# Autodesk Inventor assembly: E006_Boitier_v4
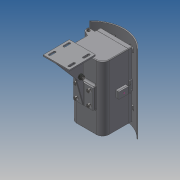
[picture p0: Inventor's stored thumbnail of the model, 180x180]
Saved by Autodesk Inventor 2021.3 (Build 253353000, 353)
## iProperties
Created: 2021-12-10
Part Number: E006_Boitier_v4
Document SubType Name: Assembly
Designer: gabri
Author: gabri
## Documents named in this file (21)
- D:\PGA\E006_Boitier_v4.iam
- D:\PGA\P037_BoitierCouvercleV4_fond.ipt
- D:\PGA\P038_BoitierCouvercleV4_couvercle.ipt
- D:\PGA\P039_BoitierCouvercleV4_capot.ipt
- D:\PGA\E003_BoitierEcran.iam
- C:\Users\gabri\Documents\Inventor\Content Center Files\R2021\en-US\AS 1474(2)\AS 1474 - M6(2).ipt
- D:\PGA\P044_SupportCaméra.ipt
- D:\PGA\P045_SupportUniversel.ipt
- C:\Users\gabri\Documents\Inventor\Content Center Files\R2021\en-US\ISO 4017(1)\ISO 4017 - M8 x 20 - ISO.ipt
- C:\Users\gabri\Documents\Inventor\Content Center Files\R2021\en-US\ISO 7040\DIEN EN ISO 7040 - M8.ipt
- D:\PGA\P046_AxeCouvercleFretté.ipt
- C:\Users\gabri\Documents\Inventor\Content Center Files\R2021\en-US\BS EN ISO 4762\BS EN ISO 4762 - M4 x 8(1).ipt
- C:\Users\gabri\Documents\Inventor\Content Center Files\R2021\en-US\DIN 6796\DIN 6796 - 4.ipt
- C:\Users\gabri\Documents\Inventor\Content Center Files\R2021\en-US\BS EN ISO 4762\BS EN ISO 4762 - M6 x 10(1).ipt
- C:\Users\gabri\Documents\Inventor\Content Center Files\R2021\en-US\BS EN ISO 4762\BS EN ISO 4762 - M5 x 16(1).ipt
- D:\PGA\P048_BoitierCouvercleV4_joint.ipt
- D:\PGA\P049_SupportTube.ipt
- D:\PGA\P050_SupportTube2.ipt
- D:\PGA\E007_Boitier_v4_moduleElectronique.iam
- D:\PGA\P051_HautGrenouillere.ipt
- D:\PGA\P052_BasGrenouillere.ipt
## Components (31 placed, 20 different names)
1. P037_BoitierCouvercleV4_fond:1 — Mate:1, Mate:2, Mate:3, Mate:5, Flush:2, Flush:3, Mate:10, Mate:11, Mate:32, Mate:33, Mate:34, Mate:35, Mate:36, Mate:37, Mate:38, Mate:39, Mate:40, Flush:4, Mate:44, Mate:58, Flush:5, Mate:59, Mate:61, Mate:64, Mate:65, Mate:69, Mate:70, Mate:71, Mate:75, Flush:7, Flush:8
2. P038_BoitierCouvercleV4_couvercle:1 — Mate:7, Mate:30, Mate:31, Insert:7, Insert:8, Insert:9, Insert:10
3. P039_BoitierCouvercleV4_capot:1 — Mate:5, Flush:2, Mate:7, Mate:30, Mate:31, Mate:72, Mate:73, Mate:74
4. E003_BoitierEcran:1 [sub-assembly] — Flush:3, Mate:10, Mate:11
5. AS 1474 (Square Nut) - Metric M6:1 — Mate:34, Mate:35
6. AS 1474 (Square Nut) - Metric M6:2 — Mate:32, Mate:33
7. AS 1474 (Square Nut) - Metric M6:3 — Mate:36, Mate:37
8. AS 1474 (Square Nut) - Metric M6:4 — Mate:38, Mate:39, Mate:41, Mate:44
9. P044_SupportCaméra:1 — Mate:40, Flush:4, Mate:41, Mate:42, Mate:43, Mate:45, Mate:46, Insert:3, Insert:4, Insert:5, Insert:6, Mate:68
10. P045_SupportUniversel:1 — Mate:42, Mate:43, Mate:48
11. ISO 4017 M8 x 20:1 — Mate:45, Mate:46, Mate:47, Mate:67
12. DIN EN ISO 7040 M8:1 — Mate:47, Mate:48
13. P046_AxeCouvercleFretté:1 — Mate:58, Flush:5, Mate:60, Mate:62
14. BS EN ISO 4762 - Metric M4 x 8:1 — Insert:2
15. BS EN ISO 4762 - Metric M4 x 8:2 — Insert:1
16. DIN 6796 4:1 — Mate:61, Mate:62, Insert:1
17. DIN 6796 4:2 — Mate:59, Mate:60, Insert:2
18. BS EN ISO 4762 - Metric M6 x 10:1 — Insert:3
19. BS EN ISO 4762 - Metric M6 x 10:2 — Insert:4
20. BS EN ISO 4762 - Metric M6 x 10:3 — Insert:5
21. BS EN ISO 4762 - Metric M6 x 10:4 — Insert:6
22. BS EN ISO 4762 - Metric M5 x 16:1 — Insert:8
23. BS EN ISO 4762 - Metric M5 x 16:2 — Insert:10
24. BS EN ISO 4762 - Metric M5 x 16:3 — Insert:9
25. BS EN ISO 4762 - Metric M5 x 16:4 — Insert:7
26. P048_BoitierCouvercleV4_joint:1 — Mate:64, Mate:65
27. P049_SupportTube:1 — Mate:66, Flush:6, Mate:67, Mate:68
28. P050_SupportTube2:1 — Mate:66, Flush:6
29. E007_Boitier_v4_moduleElectronique:1 [sub-assembly] — Mate:69, Mate:70, Mate:71
30. P051_HautGrenouillere:1 — Mate:72, Mate:73, Mate:74
31. P052_BasGrenouillere:1 — Mate:75, Flush:7, Flush:8
## Relationships (60: Mate 43, Insert 10, Flush 7)
- Mate:1: P037_BoitierCouvercleV4_fond:1
- Mate:2: P037_BoitierCouvercleV4_fond:1
- Mate:3: P037_BoitierCouvercleV4_fond:1
- Mate:5: P037_BoitierCouvercleV4_fond:1 ↔ P039_BoitierCouvercleV4_capot:1
- Flush:2: P037_BoitierCouvercleV4_fond:1 ↔ P039_BoitierCouvercleV4_capot:1
- Mate:7: P038_BoitierCouvercleV4_couvercle:1 ↔ P039_BoitierCouvercleV4_capot:1
- Flush:3: P037_BoitierCouvercleV4_fond:1 ↔ E003_BoitierEcran:1
- Mate:10: P037_BoitierCouvercleV4_fond:1 ↔ E003_BoitierEcran:1
- Mate:11: P037_BoitierCouvercleV4_fond:1 ↔ E003_BoitierEcran:1
- Mate:30: P038_BoitierCouvercleV4_couvercle:1 ↔ P039_BoitierCouvercleV4_capot:1
- Mate:31: P038_BoitierCouvercleV4_couvercle:1 ↔ P039_BoitierCouvercleV4_capot:1
- Mate:32: P037_BoitierCouvercleV4_fond:1 ↔ AS 1474 (Square Nut) - Metric M6:2
- Mate:33: P037_BoitierCouvercleV4_fond:1 ↔ AS 1474 (Square Nut) - Metric M6:2
- Mate:34: P037_BoitierCouvercleV4_fond:1 ↔ AS 1474 (Square Nut) - Metric M6:1
- Mate:35: P037_BoitierCouvercleV4_fond:1 ↔ AS 1474 (Square Nut) - Metric M6:1
- Mate:36: P037_BoitierCouvercleV4_fond:1 ↔ AS 1474 (Square Nut) - Metric M6:3
- Mate:37: P037_BoitierCouvercleV4_fond:1 ↔ AS 1474 (Square Nut) - Metric M6:3
- Mate:38: P037_BoitierCouvercleV4_fond:1 ↔ AS 1474 (Square Nut) - Metric M6:4
- Mate:39: P037_BoitierCouvercleV4_fond:1 ↔ AS 1474 (Square Nut) - Metric M6:4
- Mate:40: P037_BoitierCouvercleV4_fond:1 ↔ P044_SupportCaméra:1
- Flush:4: P037_BoitierCouvercleV4_fond:1 ↔ P044_SupportCaméra:1
- Mate:41: AS 1474 (Square Nut) - Metric M6:4 ↔ P044_SupportCaméra:1
- Mate:42: P044_SupportCaméra:1 ↔ P045_SupportUniversel:1
- Mate:43: P044_SupportCaméra:1 ↔ P045_SupportUniversel:1
- Mate:44: P037_BoitierCouvercleV4_fond:1 ↔ AS 1474 (Square Nut) - Metric M6:4
- Mate:45: P044_SupportCaméra:1 ↔ ISO 4017 M8 x 20:1
- Mate:46: P044_SupportCaméra:1 ↔ ISO 4017 M8 x 20:1
- Mate:47: ISO 4017 M8 x 20:1 ↔ DIN EN ISO 7040 M8:1
- Mate:48: P045_SupportUniversel:1 ↔ DIN EN ISO 7040 M8:1
- Mate:58: P037_BoitierCouvercleV4_fond:1 ↔ P046_AxeCouvercleFretté:1
- Flush:5: P037_BoitierCouvercleV4_fond:1 ↔ P046_AxeCouvercleFretté:1
- Mate:59: P037_BoitierCouvercleV4_fond:1 ↔ DIN 6796 4:2
- Mate:60: P046_AxeCouvercleFretté:1 ↔ DIN 6796 4:2
- Mate:61: P037_BoitierCouvercleV4_fond:1 ↔ DIN 6796 4:1
- Mate:62: P046_AxeCouvercleFretté:1 ↔ DIN 6796 4:1
- Insert:1: BS EN ISO 4762 - Metric M4 x 8:2 ↔ DIN 6796 4:1
- Insert:2: BS EN ISO 4762 - Metric M4 x 8:1 ↔ DIN 6796 4:2
- Insert:3: P044_SupportCaméra:1 ↔ BS EN ISO 4762 - Metric M6 x 10:1
- Insert:4: P044_SupportCaméra:1 ↔ BS EN ISO 4762 - Metric M6 x 10:2
- Insert:5: P044_SupportCaméra:1 ↔ BS EN ISO 4762 - Metric M6 x 10:3
- Insert:6: P044_SupportCaméra:1 ↔ BS EN ISO 4762 - Metric M6 x 10:4
- Insert:7: P038_BoitierCouvercleV4_couvercle:1 ↔ BS EN ISO 4762 - Metric M5 x 16:4
- Insert:8: P038_BoitierCouvercleV4_couvercle:1 ↔ BS EN ISO 4762 - Metric M5 x 16:1
- Insert:9: P038_BoitierCouvercleV4_couvercle:1 ↔ BS EN ISO 4762 - Metric M5 x 16:3
- Insert:10: P038_BoitierCouvercleV4_couvercle:1 ↔ BS EN ISO 4762 - Metric M5 x 16:2
- Mate:64 (1.5 mm): P037_BoitierCouvercleV4_fond:1 ↔ P048_BoitierCouvercleV4_joint:1
- Mate:65 (1.5 mm): P037_BoitierCouvercleV4_fond:1 ↔ P048_BoitierCouvercleV4_joint:1
- Mate:66: P049_SupportTube:1 ↔ P050_SupportTube2:1
- Flush:6: P049_SupportTube:1 ↔ P050_SupportTube2:1
- Mate:67: ISO 4017 M8 x 20:1 ↔ P049_SupportTube:1
- Mate:68: P044_SupportCaméra:1 ↔ P049_SupportTube:1
- Mate:69: P037_BoitierCouvercleV4_fond:1 ↔ E007_Boitier_v4_moduleElectronique:1
- Mate:70: P037_BoitierCouvercleV4_fond:1 ↔ E007_Boitier_v4_moduleElectronique:1
- Mate:71: P037_BoitierCouvercleV4_fond:1 ↔ E007_Boitier_v4_moduleElectronique:1
- Mate:72: P039_BoitierCouvercleV4_capot:1 ↔ P051_HautGrenouillere:1
- Mate:73: P039_BoitierCouvercleV4_capot:1 ↔ P051_HautGrenouillere:1
- Mate:74: P039_BoitierCouvercleV4_capot:1 ↔ P051_HautGrenouillere:1
- Mate:75: P037_BoitierCouvercleV4_fond:1 ↔ P052_BasGrenouillere:1
- Flush:7: P037_BoitierCouvercleV4_fond:1 ↔ P052_BasGrenouillere:1
- Flush:8: P037_BoitierCouvercleV4_fond:1 ↔ P052_BasGrenouillere:1
